# Autodesk Inventor assembly: CaseLeft
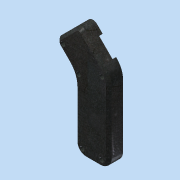
[picture p0: Inventor's stored thumbnail of the model, 180x180]
Saved by Autodesk Inventor 2015 (Build 190159000, 159)
## iProperties
Created: 2015-11-12
Part Number: CaseLeft
Document SubType Name: Assembly
Designer: Raphael
Author: Raphael
## Documents named in this file (3)
- \\psf\Home\Documents\electric-skateboard\Remote\CAD\CaseLeft.iam
- \\psf\Home\Documents\electric-skateboard\Remote\CAD\CaseLeft.ipt
- \\psf\Home\Documents\electric-skateboard\Remote\CAD\Bearing.ipt
## Components (2 placed, 2 different names)
1. CaseLeft:1 — Mate:1, Mate:2
2. Bearing:1 — Mate:1, Mate:2
## Relationships (2: Mate 2)
- Mate:1: CaseLeft:1 ↔ Bearing:1
- Mate:2: CaseLeft:1 ↔ Bearing:1
